# Autodesk Inventor assembly: MainAssembly
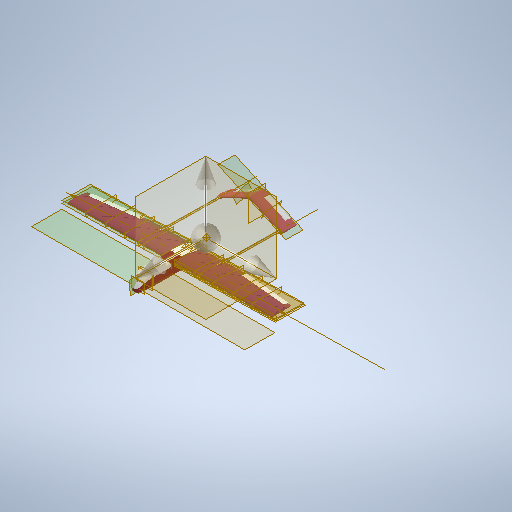
[picture p0: Inventor's stored thumbnail of the model, 512x512]
Saved by Autodesk Inventor 2026 (Build 300175050, 175E)
## iProperties
Created: 2025-08-01
Part Number: MainAssembly
Document SubType Name: Assembly
Designer: Cupri
Author: Cupri
## Documents named in this file (17)
- C:\Users\Cupri\OneDrive - University of South Carolina\Lab projects\UAV\SWIFT-UAV\System_development\Pelican\v0.2.2\MainAssembly\MainAssembly.iam
- C:\Users\Cupri\OneDrive - University of South Carolina\Lab projects\UAV\SWIFT-UAV\System_development\Pelican\v0.2.2\Parts\WingParts\WingBox.ipt
- C:\Users\Cupri\OneDrive - University of South Carolina\Lab projects\UAV\SWIFT-UAV\System_development\Pelican\v0.2.2\Parts\WingParts\WingLeft_v0.1.ipt
- C:\Users\Cupri\OneDrive - University of South Carolina\Lab projects\UAV\SWIFT-UAV\System_development\Pelican\v0.2.2\Parts\Extrusion\20x20x1295ExtrudedAluminum.ipt
- C:\Users\Cupri\OneDrive - University of South Carolina\Lab projects\UAV\SWIFT-UAV\System_development\Pelican\v0.2.2\Parts\Extrusion\20x20x800ExtrudedAluminum.ipt
- C:\Users\Cupri\OneDrive - University of South Carolina\Lab projects\UAV\SWIFT-UAV\System_development\Pelican\v0.2.2\Parts\MotorHousing.ipt
- C:\Users\Cupri\OneDrive - University of South Carolina\Lab projects\UAV\SWIFT-UAV\System_development\Pelican\v0.2.2\Parts\Motor.ipt
- C:\Users\Cupri\OneDrive - University of South Carolina\Lab projects\UAV\SWIFT-UAV\System_development\Pelican\v0.2.2\Parts\Fueselage.ipt
- C:\Users\Cupri\OneDrive - University of South Carolina\Lab projects\UAV\SWIFT-UAV\System_development\Pelican\v0.2.2\FrontCover.ipt
- C:\Users\Cupri\OneDrive - University of South Carolina\Lab projects\UAV\SWIFT-UAV\System_development\Pelican\v0.2.2\Parts\AlerionLeft.ipt
- C:\Users\Cupri\OneDrive - University of South Carolina\Lab projects\UAV\SWIFT-UAV\System_development\Pelican\v0.2.2\Parts\Extrusion\20x20x1295ExtrudedAluminum_MIR.ipt
- C:\Users\Cupri\OneDrive - University of South Carolina\Lab projects\UAV\SWIFT-UAV\System_development\Pelican\v0.2.2\Parts\AlerionLeft_MIR.ipt
- C:\Users\Cupri\OneDrive - University of South Carolina\Lab projects\UAV\SWIFT-UAV\System_development\Pelican\v0.2.2\Parts\WingParts\WingLeft_v0.1_MIR1.ipt
- C:\Users\Cupri\OneDrive - University of South Carolina\Lab projects\UAV\SWIFT-UAV\System_development\Pelican\v0.2.2\Parts\Extrusion\20x20x800ExtrudedAluminum_MIR2.ipt
- C:\Users\Cupri\OneDrive - University of South Carolina\Lab projects\UAV\SWIFT-UAV\System_development\Pelican\v0.2.2\Tail.ipt
- C:\Users\Cupri\OneDrive - University of South Carolina\Lab projects\UAV\SWIFT-UAV\System_development\Pelican\v0.2.2\Vtail.ipt
- C:\Users\Cupri\OneDrive - University of South Carolina\Lab projects\UAV\SWIFT-UAV\System_development\Pelican\v0.2.2\Vtail_MIR.ipt
## Components (16 placed, 16 different names)
1. Fueselage:1 — Mate:1, Mate:2, Flush:1, Flush:7, Mate:7, Flush:11, Mate:10, Mate:11, Flush:14
2. WingBox:1 — Mate:1, Mate:2, Mate:3, Angle:1, Flush:7
3. FrontCover:1 — Flush:1
4. 20x20x1295ExtrudedAluminum:1 — Mate:4, Mate:9
5. WingLeft_v0.1:1 — Mate:5, Angle:2, Mate:7, Mate:8, Rotational:1
6. 20x20x800ExtrudedAluminum:1 — Mate:8, Mate:9, Flush:12
7. MotorHousing:1 — Flush:11, Mate:10, Mate:11, Mate:12, Mate:13
8. Motor:1 — Mate:12, Mate:13
9. AlerionLeft:1 — Rotational:1
10. 20x20x1295ExtrudedAluminum_MIR:1 — Mate:16, Mate:19
11. WingLeft_v0.1_MIR1:1 — Mate:18, Angle:3, Mate:20, Rotational:2
12. 20x20x800ExtrudedAluminum_MIR2:1 — Mate:19, Mate:20
13. AlerionLeft_MIR:1 — Rotational:2
14. Tail:1 — Flush:13, Flush:14, Flush:15
15. Vtail:1 — Flush:15
16. Vtail_MIR:1
## Relationships (31: Mate 19, Flush 7, Angle 3, RevoluteJoint 2)
- Mate:1: Fueselage:1 ↔ WingBox:1
- Mate:2: Fueselage:1 ↔ WingBox:1
- Flush:1: Fueselage:1 ↔ FrontCover:1
- Mate:3: WingBox:1
- Angle:1 (0 deg): WingBox:1
- Mate:4: 20x20x1295ExtrudedAluminum:1
- Mate:5: WingLeft_v0.1:1
- Angle:2 (0 deg): WingLeft_v0.1:1
- Flush:7: Fueselage:1 ↔ WingBox:1
- Mate:6
- Mate:7: Fueselage:1 ↔ WingLeft_v0.1:1
- Mate:8: WingLeft_v0.1:1 ↔ 20x20x800ExtrudedAluminum:1
- Mate:9: 20x20x1295ExtrudedAluminum:1 ↔ 20x20x800ExtrudedAluminum:1
- Flush:11: Fueselage:1 ↔ MotorHousing:1
- Mate:10: Fueselage:1 ↔ MotorHousing:1
- Mate:11: Fueselage:1 ↔ MotorHousing:1
- Mate:12: MotorHousing:1 ↔ Motor:1
- Mate:13: MotorHousing:1 ↔ Motor:1
- Rotational:1 [RevoluteJoint]: WingLeft_v0.1:1 ↔ AlerionLeft:1
- Mate:15
- Mate:16: 20x20x1295ExtrudedAluminum_MIR:1
- Mate:17
- Mate:18: WingLeft_v0.1_MIR1:1
- Angle:3 (0 deg): WingLeft_v0.1_MIR1:1
- Mate:19: 20x20x1295ExtrudedAluminum_MIR:1 ↔ 20x20x800ExtrudedAluminum_MIR2:1
- Mate:20: WingLeft_v0.1_MIR1:1 ↔ 20x20x800ExtrudedAluminum_MIR2:1
- Rotational:2 [RevoluteJoint]: WingLeft_v0.1_MIR1:1 ↔ AlerionLeft_MIR:1
- Flush:12 (-100 mm): 20x20x800ExtrudedAluminum:1
- Flush:13: Tail:1
- Flush:14: Fueselage:1 ↔ Tail:1
- Flush:15: Tail:1 ↔ Vtail:1
